# Autodesk Inventor assembly: extruderAssem
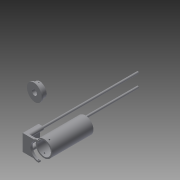
[picture p0: Inventor's stored thumbnail of the model, 180x180]
Saved by Autodesk Inventor 2015 SP2 (Build 190223200, 223)
## iProperties
Created: 2016-03-07
Part Number: extruderAssem
Document SubType Name: Assembly
Designer: marc
Author: marc
## Documents named in this file (5)
- C:\Users\marc\Documents\GitHub\Prusa_i3\Extruder\pusherDesign\extruderAssem.iam
- C:\Users\marc\Documents\GitHub\Prusa_i3\Extruder\pusherDesign\base.ipt
- C:\Users\marc\Documents\GitHub\Prusa_i3\Extruder\pusherDesign\rod.ipt
- C:\Users\marc\Documents\GitHub\Prusa_i3\Extruder\pusherDesign\CapHolder.ipt
- C:\Users\marc\Documents\GitHub\Prusa_i3\Extruder\pusherDesign\cylinder.ipt
## Components (5 placed, 4 different names)
1. base:1 — Mate:1, Mate:2, Mate:3, Cylindrical:1, Cylindrical:2, Mate:4, Mate:5, Cylindrical:3, Cylindrical:4
2. rod:1 — Cylindrical:2, Mate:5
3. rod:2 — Cylindrical:1, Mate:4
4. CapHolder:1 — Cylindrical:3
5. cylinder:1 — Cylindrical:4
## Relationships (9: Mate 5, CylindricalJoint 4)
- Mate:1: base:1
- Mate:2: base:1
- Mate:3: base:1
- Cylindrical:1: base:1 ↔ rod:2
- Cylindrical:2: base:1 ↔ rod:1
- Mate:4: base:1 ↔ rod:2
- Mate:5: base:1 ↔ rod:1
- Cylindrical:3: base:1 ↔ CapHolder:1
- Cylindrical:4: base:1 ↔ cylinder:1
